# Autodesk Inventor assembly: Assembly1
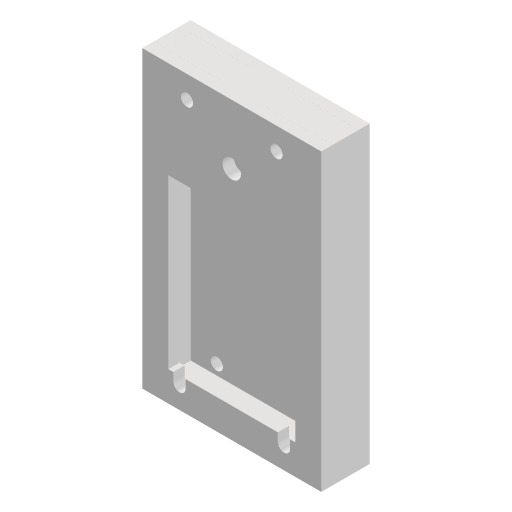
[picture p0: Inventor's stored thumbnail of the model, 512x512]
Saved by Autodesk Inventor 2023.3 (Build 273359000, 359)
## iProperties
Created: 2024-09-20
Part Number: Assembly1
Document SubType Name: Assembly
Designer: David Zindović
Author: David Zindović
## Documents named in this file (5)
- C:\Users\David Zindović\Desktop\Projekti\Darila\MyFlower\Assembly1.iam
- C:\Users\David Zindović\Desktop\Projekti\Darila\MyFlower\Bottom piece.ipt
- C:\Users\David Zindović\Desktop\Projekti\Darila\MyFlower\Side piece 2 2x.ipt
- C:\Users\David Zindović\Desktop\Projekti\Darila\MyFlower\Side piece 2x.ipt
- C:\Users\David Zindović\Desktop\Projekti\Darila\MyFlower\Top piece.ipt
## Components (6 placed, 4 different names)
1. Bottom piece:1 — Mate:1, Mate:4, Mate:5, Flush:1, Flush:2, Mate:8, Mate:9, Flush:6
2. Side piece 2 2x:1 — Flush:2, Mate:8, Mate:9, Flush:3, Flush:4, Flush:7
3. Side piece 2x:1 — Mate:1, Flush:6, Flush:7
4. Top piece:1 — Flush:3, Flush:4, Flush:5, Flush:8, Flush:9
5. Side piece 2 2x:2 — Flush:8, Flush:9, Mate:10
6. Side piece 2x:2 — Mate:4, Mate:5, Flush:1, Flush:5, Mate:10
## Relationships (15: Flush 9, Mate 6)
- Mate:1: Bottom piece:1 ↔ Side piece 2x:1
- Mate:4: Bottom piece:1 ↔ Side piece 2x:2
- Mate:5: Bottom piece:1 ↔ Side piece 2x:2
- Flush:1: Bottom piece:1 ↔ Side piece 2x:2
- Flush:2: Bottom piece:1 ↔ Side piece 2 2x:1
- Mate:8: Bottom piece:1 ↔ Side piece 2 2x:1
- Mate:9: Bottom piece:1 ↔ Side piece 2 2x:1
- Flush:3: Side piece 2 2x:1 ↔ Top piece:1
- Flush:4: Side piece 2 2x:1 ↔ Top piece:1
- Flush:5: Top piece:1 ↔ Side piece 2x:2
- Flush:6: Bottom piece:1 ↔ Side piece 2x:1
- Flush:7: Side piece 2 2x:1 ↔ Side piece 2x:1
- Flush:8: Top piece:1 ↔ Side piece 2 2x:2
- Flush:9: Top piece:1 ↔ Side piece 2 2x:2
- Mate:10: Side piece 2 2x:2 ↔ Side piece 2x:2
